# Autodesk Inventor assembly: test
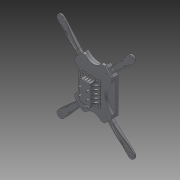
[picture p0: Inventor's stored thumbnail of the model, 180x180]
Saved by Autodesk Inventor 2015 (Build 190159000, 159)
## iProperties
Created: 2015-02-17
Part Number: test
Document SubType Name: Assembly
Designer: Piotr
Author: Piotr
## Documents named in this file (14)
- C:\Users\Piotr\Documents\Autodesk\Projects\quad v3\test.iam
- C:\Users\Piotr\Documents\Autodesk\Projects\quad v3\corps.ipt
- C:\Users\Piotr\Documents\Autodesk\Projects\quad v3\bras.ipt
- C:\Users\Piotr\Documents\Autodesk\Projects\quad v3\plaque.ipt
- C:\Users\Piotr\Documents\Autodesk\Projects\quad v3\amorti.ipt
- C:\Users\Piotr\Documents\Autodesk\Projects\quad v3\porte.ipt
- C:\Users\Piotr\Documents\Autodesk\Projects\quad v3\porte_carte.ipt
- C:\Users\Piotr\Documents\Autodesk\Projects\quad v3\pluck.ipt
- C:\Users\Piotr\Documents\Autodesk\Projects\quad v3\test\AIP\FEA\bbwit20ao.fins
- C:\Users\Piotr\Documents\Autodesk\Projects\quad v3\test\AIP\FEA\bbwit20ao.fsat
- C:\Users\Piotr\Documents\Autodesk\Projects\quad v3\test\AIP\FEA\bbwit20bk.ftes
- C:\Users\Piotr\Documents\Autodesk\Projects\quad v3\test\AIP\FEA\bbwit20bk.fwiz
- C:\Users\Piotr\Documents\Autodesk\Projects\quad v3\test\AIP\FEA\bbwit20m8.fmsh
- C:\Users\Piotr\Documents\Autodesk\Projects\quad v3\test\AIP\FEA\bbwit20m9.fres
## Components (10 placed, 7 different names)
1. corps:1 — Mate:1, Mate:2, Mate:3, Mate:4, Mate:5, Mate:6, Mate:7, Mate:8, Mate:9, Mate:10, Mate:11, Mate:12, Mate:13, Mate:14, Mate:15, Mate:16, Mate:17
2. bras:1 — Mate:1, Mate:2, Mate:3, Mate:32
3. bras:2 — Mate:11, Mate:12, Mate:13
4. bras:3 — Mate:5, Mate:6, Mate:7
5. bras:4 — Mate:8, Mate:9, Mate:10
6. plaque:1 — Mate:14, Mate:16, Mate:17, Mate:18, Mate:19, Mate:20, Mate:21, Mate:22, Mate:23, Mate:32
7. amorti:1 — Mate:18, Mate:19, Mate:20, Mate:21, Mate:22, Mate:23, Mate:24, Mate:25, Mate:26, Mate:27, Mate:28, Mate:30
8. porte:1 — Mate:24, Mate:25, Mate:29, Mate:30
9. porte_carte:1 — Mate:26, Mate:27, Mate:28, Mate:29, Mate:31
10. pluck:1 — Mate:31
## Relationships (32: Mate 32)
- Mate:1: corps:1 ↔ bras:1
- Mate:2: corps:1 ↔ bras:1
- Mate:3: corps:1 ↔ bras:1
- Mate:4: corps:1
- Mate:5: corps:1 ↔ bras:3
- Mate:6: corps:1 ↔ bras:3
- Mate:7: corps:1 ↔ bras:3
- Mate:8: corps:1 ↔ bras:4
- Mate:9: corps:1 ↔ bras:4
- Mate:10: corps:1 ↔ bras:4
- Mate:11: corps:1 ↔ bras:2
- Mate:12: corps:1 ↔ bras:2
- Mate:13: corps:1 ↔ bras:2
- Mate:14: corps:1 ↔ plaque:1
- Mate:15: corps:1
- Mate:16: corps:1 ↔ plaque:1
- Mate:17: corps:1 ↔ plaque:1
- Mate:18 (10 mm): plaque:1 ↔ amorti:1
- Mate:19: plaque:1 ↔ amorti:1
- Mate:20: plaque:1 ↔ amorti:1
- Mate:21 (10 mm): plaque:1 ↔ amorti:1
- Mate:22: plaque:1 ↔ amorti:1
- Mate:23: plaque:1 ↔ amorti:1
- Mate:24: amorti:1 ↔ porte:1
- Mate:25: amorti:1 ↔ porte:1
- Mate:26: amorti:1 ↔ porte_carte:1
- Mate:27: amorti:1 ↔ porte_carte:1
- Mate:28: amorti:1 ↔ porte_carte:1
- Mate:29: porte:1 ↔ porte_carte:1
- Mate:30: amorti:1 ↔ porte:1
- Mate:31: porte_carte:1 ↔ pluck:1
- Mate:32: bras:1 ↔ plaque:1
## Named parameters: sa_0 = 1.5e-12, sa_1 = 10000, sa_2 = -1.8e-12
note: some values were not read from the file. Shown as the stored number, unit unknown: "sa_0", "sa_1", "sa_2".
